# Autodesk Inventor assembly: Quad Assy
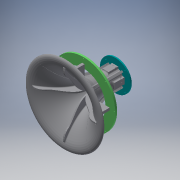
[picture p0: Inventor's stored thumbnail of the model, 180x180]
Saved by Autodesk Inventor 2016 SP1 (Build 200210100, 210)
## iProperties
Created: 2015-10-31
Part Number: Quad Assy
Description: STEP AP214
Document SubType Name: Assembly
Designer: Dave
Sending System: SolidWorks 2003240
Preprocessor: SwSTEP 2.0
Title: Quad Assy.STEP
Revision Number: ANY
## Documents named in this file (10)
- C:\Users\ddeboer\Desktop\leuschner-cad\feed.iam
- C:\Users\ddeboer\Desktop\leuschner-cad\connector.ipt
- C:\Users\ddeboer\Desktop\leuschner-cad\1.15 Quadrent 1.ipt
- C:\Users\ddeboer\Desktop\leuschner-cad\Berkeley ring.ipt
- C:\Users\ddeboer\Desktop\leuschner-cad\1.15 Quadrent 1_Default .437.ipt
- C:\Users\ddeboer\Desktop\leuschner-cad\Horn Base.ipt
- C:\Users\ddeboer\Desktop\leuschner-cad\1.15 Quadrent 1_Opposite.ipt
- C:\Users\ddeboer\Desktop\leuschner-cad\1.15 Quadrent 1_Opposide 437.ipt
- C:\Users\ddeboer\Desktop\leuschner-cad\pin.ipt
- C:\Users\ddeboer\Desktop\leuschner-cad\mountingRing.ipt
## Components (13 placed, 13 different names)
1. connector_1
2. 1.15 Quadrent 1_2 — Insert:1
3. Berkeley ring_3
4. Berkeley ring_5
5. 1.15 Quadrent 1_Default .437_6
6. Horn Base_7
7. Berkeley ring_8
8. 1.15 Quadrent 1_Opposite_9
9. Berkeley ring_10
10. connector_11
11. 1.15 Quadrent 1_Opposide 437_12
12. pin_13
13. mountingRing:1 — Insert:1
## Relationships (1: Insert 1)
- Insert:1: 1.15 Quadrent 1_2 ↔ mountingRing:1
